# Autodesk Inventor assembly: McCrea_pasy_zlozene_walle_MIR
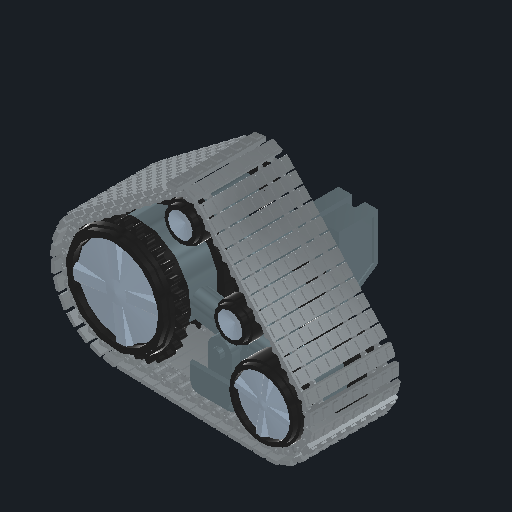
[picture p0: Inventor's stored thumbnail of the model, 512x512]
Saved by Autodesk Inventor 2022 (Build 260153000, 153)
## iProperties
Created: 2022-01-09
Part Number: McCrea_pasy_zlozene_walle_MIR
Document SubType Name: Assembly
Designer: MatusBarany
Author: MatusBarany
## Documents named in this file (12)
- C:\Users\MatusBarany\Documents\Inventor\wall-e\matus\McCrea_pasy_zlozene_walle_MIR.iam
- C:\Users\MatusBarany\Documents\Inventor\wall-e\matus\McCrea_chrbat_walle_MIR.ipt
- C:\Users\MatusBarany\Documents\Inventor\wall-e\matus\McCrea_male_koleso_walle_MIR.ipt
- C:\Users\MatusBarany\Documents\Inventor\wall-e\matus\McCrea_polspojka_stredne_koleso_walle_MIR.ipt
- C:\Users\MatusBarany\Documents\Inventor\wall-e\matus\McCrea_polspojka_velke_koleso_walle_MIR.ipt
- C:\Users\MatusBarany\Documents\Inventor\wall-e\matus\McCrea_spojka_male_koleso_walle_MIR.ipt
- C:\Users\MatusBarany\Documents\Inventor\wall-e\matus\McCrea_spojka_pasy_telo_walle_MIR.ipt
- C:\Users\MatusBarany\Documents\Inventor\wall-e\matus\McCrea_velke_koleso_walle_MIR.ipt
- C:\Users\MatusBarany\Documents\Inventor\wall-e\matus\McCrea_stredne_koleso_walle_MIR.ipt
- C:\Users\MatusBarany\Documents\Inventor\wall-e\matus\McCrea_uchytka_walle_MIR.ipt
- C:\Users\Public\Documents\Autodesk\Inventor 2022\McCrea_draha_walle_MIR.ipt
- C:\Users\MatusBarany\Documents\Inventor\wall-e\matus\McCrea_diel_retaze_walle_MIR.ipt
## Components (68 placed, 11 different names)
1. McCrea_chrbat_walle_MIR:1 — Mate:6, Mate:5, Mate:1, Mate:4, Mate:3, Mate:2, Rotational:1
2. McCrea_male_koleso_walle_MIR:1 — Rigid:4
3. McCrea_polspojka_stredne_koleso_walle_MIR:1 — Mate:9, Flush:1, Mate:8, Rigid:3, Rigid:2
4. McCrea_polspojka_velke_koleso_walle_MIR:1 — Mate:9, Flush:1, Mate:8, Mate:7, Rigid:1, Rotational:2, Cylindrical:1
5. McCrea_spojka_male_koleso_walle_MIR:1 — Rigid:4, Rotational:1, Rigid:7, Rigid:6, Rigid:5
6. McCrea_spojka_pasy_telo_walle_MIR:1 — Mate:6, Mate:5, Mate:1
7. McCrea_velke_koleso_walle_MIR:1 — Rigid:1
8. McCrea_velke_koleso_walle_MIR:2 — Flush:2, Rotational:2
9. McCrea_stredne_koleso_walle_MIR:1 — Rigid:3
10. McCrea_uchytka_walle_MIR:1 — Mate:7, Mate:4, Mate:3, Mate:2, Cylindrical:1
11. McCrea_male_koleso_walle_MIR:2 — Rigid:7
12. McCrea_stredne_koleso_walle_MIR:2 — Rigid:2
13. McCrea_male_koleso_walle_MIR:3 — Rigid:6
14. McCrea_male_koleso_walle_MIR:4 — Rigid:5
15. McCrea_draha_walle_MIR:1 — Mate:12, Mate:11, Mate:10, Flush:2
16. McCrea_diel_retaze_walle_MIR:1 — Mate:12, Mate:11, Mate:10
17. McCrea_diel_retaze_walle_MIR:2
18. McCrea_diel_retaze_walle_MIR:3
19. McCrea_diel_retaze_walle_MIR:4
20. McCrea_diel_retaze_walle_MIR:5
21. McCrea_diel_retaze_walle_MIR:6
22. McCrea_diel_retaze_walle_MIR:7
23. McCrea_diel_retaze_walle_MIR:8
24. McCrea_diel_retaze_walle_MIR:9
25. McCrea_diel_retaze_walle_MIR:10
26. McCrea_diel_retaze_walle_MIR:11
27. McCrea_diel_retaze_walle_MIR:12
28. McCrea_diel_retaze_walle_MIR:13
29. McCrea_diel_retaze_walle_MIR:14
30. McCrea_diel_retaze_walle_MIR:15
31. McCrea_diel_retaze_walle_MIR:16
32. McCrea_diel_retaze_walle_MIR:17
33. McCrea_diel_retaze_walle_MIR:18
34. McCrea_diel_retaze_walle_MIR:19
35. McCrea_diel_retaze_walle_MIR:20
36. McCrea_diel_retaze_walle_MIR:21
37. McCrea_diel_retaze_walle_MIR:22
38. McCrea_diel_retaze_walle_MIR:23
39. McCrea_diel_retaze_walle_MIR:24
40. McCrea_diel_retaze_walle_MIR:25
41. McCrea_diel_retaze_walle_MIR:26
42. McCrea_diel_retaze_walle_MIR:27
43. McCrea_diel_retaze_walle_MIR:28
44. McCrea_diel_retaze_walle_MIR:29
45. McCrea_diel_retaze_walle_MIR:30
46. McCrea_diel_retaze_walle_MIR:31
47. McCrea_diel_retaze_walle_MIR:32
48. McCrea_diel_retaze_walle_MIR:33
49. McCrea_diel_retaze_walle_MIR:34
50. McCrea_diel_retaze_walle_MIR:35
51. McCrea_diel_retaze_walle_MIR:36
52. McCrea_diel_retaze_walle_MIR:37
53. McCrea_diel_retaze_walle_MIR:38
54. McCrea_diel_retaze_walle_MIR:39
55. McCrea_diel_retaze_walle_MIR:40
56. McCrea_diel_retaze_walle_MIR:41
57. McCrea_diel_retaze_walle_MIR:42
58. McCrea_diel_retaze_walle_MIR:43
59. McCrea_diel_retaze_walle_MIR:44
60. McCrea_diel_retaze_walle_MIR:45
61. McCrea_diel_retaze_walle_MIR:46
62. McCrea_diel_retaze_walle_MIR:47
63. McCrea_diel_retaze_walle_MIR:48
64. McCrea_diel_retaze_walle_MIR:49
65. McCrea_diel_retaze_walle_MIR:50
66. McCrea_diel_retaze_walle_MIR:51
67. McCrea_diel_retaze_walle_MIR:52
68. McCrea_diel_retaze_walle_MIR:53
## Relationships (24: Mate 13, WeldJoint 7, RevoluteJoint 2, Flush 1, CylindricalJoint 1)
- Mate:9: McCrea_polspojka_stredne_koleso_walle_MIR:1 ↔ McCrea_polspojka_velke_koleso_walle_MIR:1
- Flush:1: McCrea_polspojka_stredne_koleso_walle_MIR:1 ↔ McCrea_polspojka_velke_koleso_walle_MIR:1
- Mate:8: McCrea_polspojka_stredne_koleso_walle_MIR:1 ↔ McCrea_polspojka_velke_koleso_walle_MIR:1
- Mate:6: McCrea_chrbat_walle_MIR:1 ↔ McCrea_spojka_pasy_telo_walle_MIR:1
- Mate:5: McCrea_chrbat_walle_MIR:1 ↔ McCrea_spojka_pasy_telo_walle_MIR:1
- Mate:1: McCrea_chrbat_walle_MIR:1 ↔ McCrea_spojka_pasy_telo_walle_MIR:1
- Mate:7: McCrea_polspojka_velke_koleso_walle_MIR:1 ↔ McCrea_uchytka_walle_MIR:1
- Mate:4: McCrea_chrbat_walle_MIR:1 ↔ McCrea_uchytka_walle_MIR:1
- Mate:3: McCrea_chrbat_walle_MIR:1 ↔ McCrea_uchytka_walle_MIR:1
- Mate:2: McCrea_chrbat_walle_MIR:1 ↔ McCrea_uchytka_walle_MIR:1
- Mate:12: McCrea_draha_walle_MIR:1 ↔ McCrea_diel_retaze_walle_MIR:1
- Mate:11: McCrea_draha_walle_MIR:1 ↔ McCrea_diel_retaze_walle_MIR:1
- Mate:10: McCrea_draha_walle_MIR:1 ↔ McCrea_diel_retaze_walle_MIR:1
- Flush:2 [Mate] (-1.4986 mm): McCrea_velke_koleso_walle_MIR:2 ↔ McCrea_draha_walle_MIR:1
- Rigid:4 [WeldJoint]: McCrea_male_koleso_walle_MIR:1 ↔ McCrea_spojka_male_koleso_walle_MIR:1
- Rotational:1 [RevoluteJoint]: McCrea_chrbat_walle_MIR:1 ↔ McCrea_spojka_male_koleso_walle_MIR:1
- Rigid:1 [WeldJoint]: McCrea_polspojka_velke_koleso_walle_MIR:1 ↔ McCrea_velke_koleso_walle_MIR:1
- Rotational:2 [RevoluteJoint]: McCrea_polspojka_velke_koleso_walle_MIR:1 ↔ McCrea_velke_koleso_walle_MIR:2
- Rigid:3 [WeldJoint]: McCrea_polspojka_stredne_koleso_walle_MIR:1 ↔ McCrea_stredne_koleso_walle_MIR:1
- Cylindrical:1: McCrea_polspojka_velke_koleso_walle_MIR:1 ↔ McCrea_uchytka_walle_MIR:1
- Rigid:7 [WeldJoint]: McCrea_spojka_male_koleso_walle_MIR:1 ↔ McCrea_male_koleso_walle_MIR:2
- Rigid:2 [WeldJoint]: McCrea_polspojka_stredne_koleso_walle_MIR:1 ↔ McCrea_stredne_koleso_walle_MIR:2
- Rigid:6 [WeldJoint]: McCrea_spojka_male_koleso_walle_MIR:1 ↔ McCrea_male_koleso_walle_MIR:3
- Rigid:5 [WeldJoint]: McCrea_spojka_male_koleso_walle_MIR:1 ↔ McCrea_male_koleso_walle_MIR:4
